# Autodesk Inventor assembly: Electromagnet
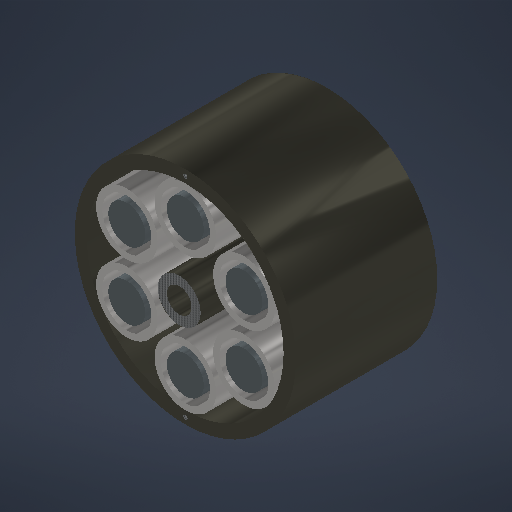
[picture p0: Inventor's stored thumbnail of the model, 512x512]
Saved by Autodesk Inventor 2026.3 (Build 303398000, 398)
## iProperties
Created: 2026-07-22
Part Number: Electromagnet
Document SubType Name: Assembly
Designer: matot
Author: matot
## Documents named in this file (4)
- C:\Users\matot\OneDrive - Stellenbosch University\2026\MechatronicsProject478\Building the joint\Joint Assembly\Electromagnet.iam
- C:\Users\matot\OneDrive - Stellenbosch University\2026\MechatronicsProject478\Building the joint\Joint Assembly\Solenoid core.ipt
- C:\Users\matot\OneDrive - Stellenbosch University\2026\MechatronicsProject478\Building the joint\Joint Assembly\Solenoid Yoke.ipt
- C:\Users\matot\OneDrive - Stellenbosch University\2026\MechatronicsProject478\Building the joint\Joint Assembly\Electromagnet cover.ipt
## Components (13 placed, 3 different names)
1. Solenoid core:1 — Insert:4
2. Solenoid core:2 — Insert:2
3. Solenoid core:3 — Insert:3
4. Solenoid core:4 — Insert:5
5. Solenoid core:5 — Insert:6
6. Solenoid core:6 — Insert:1
7. Solenoid Yoke:1 — Insert:2, Insert:9
8. Solenoid Yoke:2 — Insert:3, Insert:8
9. Solenoid Yoke:3 — Insert:4, Insert:12
10. Solenoid Yoke:4 — Insert:5, Insert:11
11. Solenoid Yoke:5 — Insert:6, Insert:7
12. Solenoid Yoke:6 — Insert:1, Insert:10
13. Electromagnet cover:1 — Insert:7, Insert:8, Insert:9, Insert:10, Insert:11, Insert:12
## Relationships (12: Insert 12)
- Insert:1: Solenoid core:6 ↔ Solenoid Yoke:6
- Insert:2: Solenoid core:2 ↔ Solenoid Yoke:1
- Insert:3: Solenoid core:3 ↔ Solenoid Yoke:2
- Insert:4: Solenoid core:1 ↔ Solenoid Yoke:3
- Insert:5: Solenoid core:4 ↔ Solenoid Yoke:4
- Insert:6: Solenoid core:5 ↔ Solenoid Yoke:5
- Insert:7: Solenoid Yoke:5 ↔ Electromagnet cover:1
- Insert:8: Solenoid Yoke:2 ↔ Electromagnet cover:1
- Insert:9: Solenoid Yoke:1 ↔ Electromagnet cover:1
- Insert:10: Solenoid Yoke:6 ↔ Electromagnet cover:1
- Insert:11: Solenoid Yoke:4 ↔ Electromagnet cover:1
- Insert:12: Solenoid Yoke:3 ↔ Electromagnet cover:1
